# Autodesk Inventor assembly: Car_Assembly
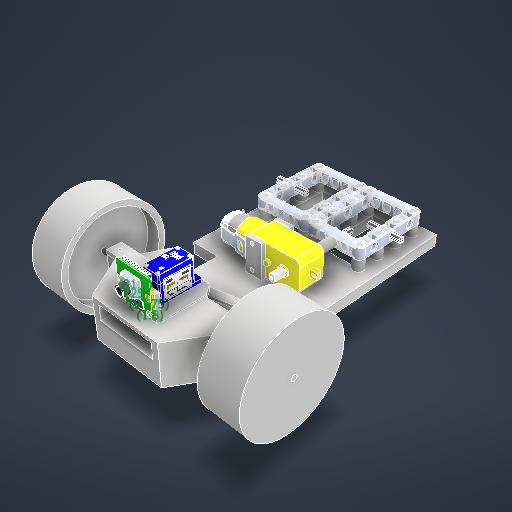
[picture p0: Inventor's stored thumbnail of the model, 512x512]
Saved by Autodesk Inventor 2025 (Build 290162000, 162)
## iProperties
Created: 2024-05-24
Part Number: Car_Assembly
Document SubType Name: Assembly
Designer: Garfieldcmix
Author: Garfieldcmix
## Documents named in this file (16)
- C:\Users\chaya\Desktop\WRO-2024-CAD\Car_Assembly.iam
- C:\Users\chaya\Desktop\WRO-2024-CAD\SG90 - Micro Servo 9g - Tower Pro\SG90 - Micro Servo 9g - Tower Pro.iam
- C:\Users\chaya\Desktop\WRO-2024-CAD\Front_Bridge.ipt
- C:\Users\chaya\Desktop\WRO-2024-CAD\SG90 - Micro Servo 9g - Tower Pro\SG90 - Micro Servo 9g - Tower Pro.2.ipt
- C:\Users\chaya\Desktop\WRO-2024-CAD\Front_Wheel_Anchor.ipt
- C:\Users\chaya\Desktop\WRO-2024-CAD\Front_Wheel_Anchor_MIR.ipt
- C:\Users\chaya\Desktop\WRO-2024-CAD\Wheel.ipt
- C:\Users\chaya\Desktop\WRO-2024-CAD\Wheel_MIR.ipt
- C:\Users\chaya\Desktop\WRO-2024-CAD\Servo_Steering_Linkage.ipt
- C:\Users\chaya\Desktop\WRO-2024-CAD\Servo_Steering_Linkage_MIR.ipt
- C:\Users\chaya\Desktop\WRO-2024-CAD\Pi camera module3\Pi camera module3.ipt
- C:\Users\chaya\Desktop\WRO-2024-CAD\4519 DkStone Technic Axle 3\4519 DkStone Technic Axle 3.ipt
- C:\Users\chaya\Desktop\WRO-2024-CAD\Lego Beam Fram 5x7 (64179)\Lego Beam Fram 5x7 (64179).ipt
- C:\Users\chaya\Desktop\WRO-2024-CAD\TT Motor\TT Motor.ipt
- C:\Users\chaya\Desktop\WRO-2024-CAD\Lower_Chassis.ipt
- C:\Users\chaya\Desktop\WRO-2024-CAD\Motor_Lego_Axle_Connector.ipt
## Components (18 placed, 18 different names)
1. Front_Bridge:1 — Mate:1, Mate:16, Mate:18, Mate:19, Mate:21, Mate:22, Angle:1, Mate:32, Mate:33, Mate:34, Mate:35, Mate:36, Mate:38, Mate:39, Mate:40, Mate:41, Mate:42
2. Pi camera module3:1 — Mate:32, Mate:33, Mate:34, Mate:35, Mate:36
3. Lower_Chassis:1 — Mate:38, Mate:39, Mate:40, Mate:41, Mate:42, Mate:43, Mate:44, Mate:45, Mate:46, Mate:47, Mate:48, Mate:56, Mate:57
4. Left_Lego_Beam_Frame — Mate:37, Mate:43, Mate:44, Mate:45, Mate:50, Mate:55
5. Right_Lego_Beam_Frame — Mate:46, Mate:47, Mate:48, Mate:49
6. Left_Lego_Wheel_Axle — Mate:37
7. Right_Lego_Wheel_Axle — Mate:49
8. Lego_Driving_Shaft_Axle — Mate:50, Mate:53, Mate:54
9. TT Motor:1 — Mate:51, Mate:52, Mate:56, Mate:57
10. Motor_Lego_Axle_Connector:1 — Mate:51, Mate:52, Mate:53, Mate:54, Mate:55
11. Left_Front_Wheel_Anchor — Mate:18, Mate:19, Mate:20, Flush:1, Mate:24, Mate:26, Angle:1
12. Left_Front_Wheel — Mate:20, Flush:1
13. Right_Front_Wheel_Anchor — Mate:21, Mate:22, Mate:23, Flush:2, Mate:28, Mate:29
14. Right_Front_Wheel — Mate:23, Flush:2
15. Left_Servo_Steering_Linkage — Mate:24, Mate:25, Mate:26, Mate:27
16. Right_Servo_Steering_Linkage — Mate:28, Mate:31, Mate:29, Mate:30
17. SG90_Servo [sub-assembly] — Mate:1, Mate:16, Mate:2, Mate:17
18. Servo_Arm — Mate:2, Mate:17, Mate:25, Mate:27, Mate:30, Mate:31
## Relationships (47: Mate 44, Flush 2, Angle 1)
- Mate:1: Front_Bridge:1 ↔ SG90_Servo
- Mate:16: Front_Bridge:1 ↔ SG90_Servo
- Mate:2: SG90_Servo ↔ Servo_Arm
- Mate:17: SG90_Servo ↔ Servo_Arm
- Mate:18: Front_Bridge:1 ↔ Left_Front_Wheel_Anchor
- Mate:19: Front_Bridge:1 ↔ Left_Front_Wheel_Anchor
- Mate:20: Left_Front_Wheel_Anchor ↔ Left_Front_Wheel
- Flush:1: Left_Front_Wheel_Anchor ↔ Left_Front_Wheel
- Mate:21: Front_Bridge:1 ↔ Right_Front_Wheel_Anchor
- Mate:22: Front_Bridge:1 ↔ Right_Front_Wheel_Anchor
- Mate:23: Right_Front_Wheel_Anchor ↔ Right_Front_Wheel
- Flush:2: Right_Front_Wheel_Anchor ↔ Right_Front_Wheel
- Mate:24: Left_Front_Wheel_Anchor ↔ Left_Servo_Steering_Linkage
- Mate:25: Left_Servo_Steering_Linkage ↔ Servo_Arm
- Mate:26: Left_Front_Wheel_Anchor ↔ Left_Servo_Steering_Linkage
- Angle:1 (145 deg): Front_Bridge:1 ↔ Left_Front_Wheel_Anchor
- Mate:27: Left_Servo_Steering_Linkage ↔ Servo_Arm
- Mate:28: Right_Front_Wheel_Anchor ↔ Right_Servo_Steering_Linkage
- Mate:31: Right_Servo_Steering_Linkage ↔ Servo_Arm
- Mate:29: Right_Front_Wheel_Anchor ↔ Right_Servo_Steering_Linkage
- Mate:30: Right_Servo_Steering_Linkage ↔ Servo_Arm
- Mate:32: Front_Bridge:1 ↔ Pi camera module3:1
- Mate:33: Front_Bridge:1 ↔ Pi camera module3:1
- Mate:34: Front_Bridge:1 ↔ Pi camera module3:1
- Mate:35: Front_Bridge:1 ↔ Pi camera module3:1
- Mate:36: Front_Bridge:1 ↔ Pi camera module3:1
- Mate:37: Left_Lego_Beam_Frame ↔ Left_Lego_Wheel_Axle
- Mate:38: Front_Bridge:1 ↔ Lower_Chassis:1
- Mate:39: Front_Bridge:1 ↔ Lower_Chassis:1
- Mate:40: Front_Bridge:1 ↔ Lower_Chassis:1
- Mate:41: Front_Bridge:1 ↔ Lower_Chassis:1
- Mate:42: Front_Bridge:1 ↔ Lower_Chassis:1
- Mate:43: Lower_Chassis:1 ↔ Left_Lego_Beam_Frame
- Mate:44: Lower_Chassis:1 ↔ Left_Lego_Beam_Frame
- Mate:45: Lower_Chassis:1 ↔ Left_Lego_Beam_Frame
- Mate:46: Lower_Chassis:1 ↔ Right_Lego_Beam_Frame
- Mate:47: Lower_Chassis:1 ↔ Right_Lego_Beam_Frame
- Mate:48: Lower_Chassis:1 ↔ Right_Lego_Beam_Frame
- Mate:49: Right_Lego_Beam_Frame ↔ Right_Lego_Wheel_Axle
- Mate:50: Left_Lego_Beam_Frame ↔ Lego_Driving_Shaft_Axle
- Mate:51: TT Motor:1 ↔ Motor_Lego_Axle_Connector:1
- Mate:52: TT Motor:1 ↔ Motor_Lego_Axle_Connector:1
- Mate:53: Lego_Driving_Shaft_Axle ↔ Motor_Lego_Axle_Connector:1
- Mate:54: Lego_Driving_Shaft_Axle ↔ Motor_Lego_Axle_Connector:1
- Mate:55: Left_Lego_Beam_Frame ↔ Motor_Lego_Axle_Connector:1
- Mate:56: Lower_Chassis:1 ↔ TT Motor:1
- Mate:57: Lower_Chassis:1 ↔ TT Motor:1
